# Autodesk Inventor assembly: Сальник
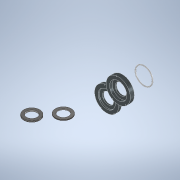
[picture p0: Inventor's stored thumbnail of the model, 180x180]
Saved by Autodesk Inventor 2021 (Build 250183000, 183)
## iProperties
Created: 2020-12-13
Part Number: Сальник
Document SubType Name: Assembly
Designer: Тимоха
Author: Тимоха
## Documents named in this file (8)
- C:\Users\Тимоха\Desktop\КР Компрессор\compressor\Сальник.iam
- C:\Users\Тимоха\Desktop\КР Компрессор\compressor\Дроссельное кольцо.ipt
- C:\Users\Тимоха\Desktop\КР Компрессор\compressor\Кольцо сальника.ipt
- C:\Users\Тимоха\Desktop\КР Компрессор\compressor\Корпус дросселя.ipt
- C:\Users\Тимоха\Desktop\КР Компрессор\compressor\Корпус сальника.ipt
- C:\Users\Тимоха\Desktop\КР Компрессор\compressor\Уплотнительное кольцо.ipt
- C:\Users\Тимоха\Desktop\КР Компрессор\compressor\Пружина дросселя.ipt
- C:\Users\Тимоха\Desktop\КР Компрессор\compressor\Пружина сальника.ipt
## Components (7 placed, 7 different names)
1. Дроссельное кольцо:1 — Жесткий:1
2. Кольцо сальника:1 — Жесткий:2
3. Корпус дросселя:1
4. Корпус сальника:1
5. Уплотнительное кольцо:1
6. Пружина дросселя:1 — Жесткий:1
7. Пружина сальника:1 — Жесткий:2
## Relationships (2: WeldJoint 2)
- Жесткий:1 [WeldJoint]: Дроссельное кольцо:1 ↔ Пружина дросселя:1
- Жесткий:2 [WeldJoint]: Кольцо сальника:1 ↔ Пружина сальника:1
